# Autodesk Inventor assembly: Capstone Placer
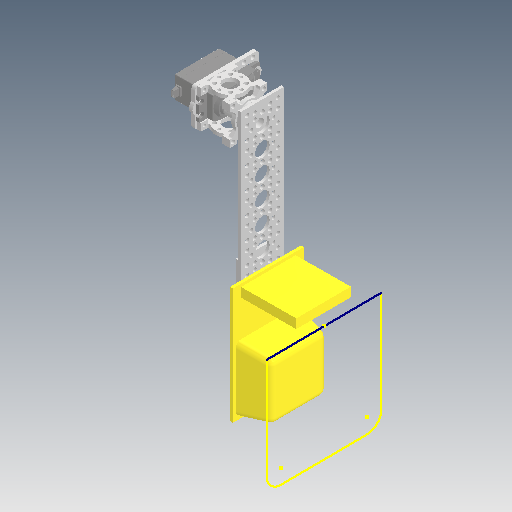
[picture p0: Inventor's stored thumbnail of the model, 512x512]
Saved by Autodesk Inventor 2020 (Build 240168000, 168)
## iProperties
Created: 2020-01-29
Part Number: Capstone Placer
Document SubType Name: Assembly
Designer: ball
Author: ball
## Documents named in this file (5)
- C:\FTC\FTC8863CAD\2019 Robot\Delivery\Capstone\Capstone Placer.iam
- C:\FTC\FTC8863CAD\2019 Robot\Collection\servo block assembly.iam
- C:\FTC\FTC8863CAD\2019 Robot\Collection\8863 capstone.ipt
- C:\FTC\FTC8863CAD\Actobotics\585 parts\585723.ipt
- C:\FTC\FTC8863CAD\Actobotics\585 parts\585506.ipt
## Components (4 placed, 4 different names)
1. servo block assembly:1 [sub-assembly]
2. 8863 capstone:1
3. 585723:1
4. 585506:1
## Relationships (7: Mate 6, Flush 1)
- [Mate]: servo block assembly:1 ↔ 585723:1
- [Mate]: 585723:1 ↔ 585506:1
- [Flush]: 585723:1 ↔ 585506:1
- [Mate]: 585723:1 ↔ 585506:1
- [Mate]: 8863 capstone:1 ↔ 585506:1
- [Mate]: 8863 capstone:1 ↔ 585506:1
- [Mate]: servo block assembly:1 ↔ 585723:1
